# Autodesk Inventor assembly: fileSocketHanger
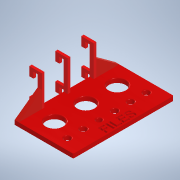
[picture p0: Inventor's stored thumbnail of the model, 180x180]
Saved by Autodesk Inventor 2021 (Build 250183000, 183)
## iProperties
Created: 2020-03-15
Part Number: fileSocketHanger
Document SubType Name: Assembly
Designer: robst
Author: robst
## Documents named in this file (4)
- C:\git\CAD-Development\robSteele\HouseProjects\Garage\Ikea\fileSocketHanger.iam
- C:\git\CAD-Development\robSteele\HouseProjects\Garage\Ikea\threeStartConfigurationV01.ipt
- C:\git\CAD-Development\robSteele\HouseProjects\Garage\Ikea\plateForFileSet.ipt
- C:\git\CAD-Development\robSteele\HouseProjects\Garage\Ikea\supportForFileHanger.ipt
## Components (3 placed, 3 different names)
1. threeStartConfigurationV01:1 — Mate:1, Flush:1, Flush:2, Flush:3, Flush:4
2. plateForFileSet:1 — Mate:1, Flush:1, Flush:2
3. supportForFileHanger:1 — Flush:3, Flush:4
## Relationships (5: Flush 4, Mate 1)
- Mate:1: threeStartConfigurationV01:1 ↔ plateForFileSet:1
- Flush:1: threeStartConfigurationV01:1 ↔ plateForFileSet:1
- Flush:2: threeStartConfigurationV01:1 ↔ plateForFileSet:1
- Flush:3: threeStartConfigurationV01:1 ↔ supportForFileHanger:1
- Flush:4: threeStartConfigurationV01:1 ↔ supportForFileHanger:1
